# Autodesk Inventor assembly: 헤드 조립
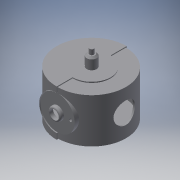
[picture p0: Inventor's stored thumbnail of the model, 180x180]
Saved by Autodesk Inventor 2018 (Build 220112000, 112)
## iProperties
Created: 2018-04-19
Part Number: 헤드 조립
Material: 일반
Document SubType Name: Assembly
Designer: CK
Author: CK
## Documents named in this file (3)
- C:\Users\CK\Desktop\캡스톤\헤드 조립.iam
- C:\Users\CK\Desktop\캡스톤\헤드(상).ipt
- C:\Users\CK\Desktop\캡스톤\헤드(하).ipt
## Components (2 placed, 2 different names)
1. 헤드(상):1 — 메이트:2, 메이트:3, 메이트:4
2. 헤드(하):1 — 메이트:2, 메이트:3, 메이트:4
## Relationships (3: Mate 3)
- 메이트:2 [Mate]: 헤드(상):1 ↔ 헤드(하):1
- 메이트:3 [Mate]: 헤드(상):1 ↔ 헤드(하):1
- 메이트:4 [Mate]: 헤드(상):1 ↔ 헤드(하):1
